# Autodesk Inventor assembly: Manipulator
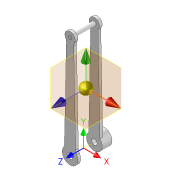
[picture p0: Inventor's stored thumbnail of the model, 180x180]
Saved by Autodesk Inventor 2020 (Build 240168000, 168)
## iProperties
Created: 2020-03-27
Part Number: Manipulator
Document SubType Name: Assembly
Designer: JakubTomaszewski
Mass: 30.4924 g
Surface Area: 141.041 cm^2
Volume: 22.9643 cm^3
Density: 1.32782 g/cm^3
Author: JakubTomaszewski
## Documents named in this file (4)
- C:\Users\JakubTomaszewski\Documents\Inventor\Manipulator\DrugieOgniwo.iam
- C:\Users\JakubTomaszewski\Documents\Inventor\Manipulator\Ogniwo1.1.ipt
- C:\Users\JakubTomaszewski\Documents\Inventor\Manipulator\Ogniwo1.2.ipt
- C:\Users\JakubTomaszewski\Documents\Inventor\Manipulator\Ogniwo1_lacznik.ipt
## Components (3 placed, 3 different names)
1. Ogniwo1.1:1 — Lącznik1.1, Równoległe:1, Równoległe:2, Równoległe:3
2. Ogniwo1.2:1 — Lącznik1.2
3. Ogniwo1_lacznik:1 — Lącznik1.2, Lącznik1.1
## Relationships (5: Flush 3, WeldJoint 2)
- Lącznik1.2 [WeldJoint]: Ogniwo1.2:1 ↔ Ogniwo1_lacznik:1
- Lącznik1.1 [WeldJoint]: Ogniwo1.1:1 ↔ Ogniwo1_lacznik:1
- Równoległe:1 [Flush]: Ogniwo1.1:1
- Równoległe:2 [Flush]: Ogniwo1.1:1
- Równoległe:3 [Flush]: Ogniwo1.1:1
